# Autodesk Inventor assembly: test_bench_1
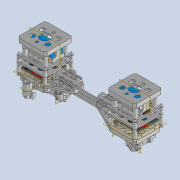
[picture p0: Inventor's stored thumbnail of the model, 180x180]
Saved by Autodesk Inventor 2020 (Build 240168000, 168)
## iProperties
Created: 2022-01-22
Part Number: test_bench_1
Document SubType Name: Assembly
Designer: Shuang Peng
Author: Shuang Peng
## Documents named in this file (4)
- D:\projects-3\soft module robot\hardware\diff module 3\test_bench_1.iam
- D:\projects-3\soft module robot\hardware\diff module 3\base_ass_3.iam
- D:\projects-3\soft module robot\hardware\diff module 3\test_bridge_1.ipt
- D:\projects-3\soft module robot\hardware\diff module 3\test_bridge_2.ipt
## Components (4 placed, 3 different names)
1. base_ass_3:1 [sub-assembly] — Angle:1, Flush:1, Mate:1, Flush:2, Flush:3
2. base_ass_3:2 [sub-assembly] — Flush:1, Mate:1, Flush:2, Flush:4
3. test_bridge_1:1 — Flush:3
4. test_bridge_2:1 — Flush:4
## Relationships (6: Flush 4, Angle 1, Mate 1)
- Angle:1 (180 deg): base_ass_3:1
- Flush:1: base_ass_3:1 ↔ base_ass_3:2
- Mate:1 (100 mm): base_ass_3:1 ↔ base_ass_3:2
- Flush:2: base_ass_3:1 ↔ base_ass_3:2
- Flush:3: base_ass_3:1 ↔ test_bridge_1:1
- Flush:4: base_ass_3:2 ↔ test_bridge_2:1
